# Autodesk Inventor assembly: WheelAssembly
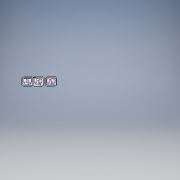
[picture p0: Inventor's stored thumbnail of the model, 180x180]
Saved by Autodesk Inventor 2016 (Build 200138000, 138)
## iProperties
Created: 2016-09-10
Part Number: WheelAssembly
Document SubType Name: Assembly
Designer: RoboticsUser
Author: RoboticsUser
## Documents named in this file (10)
- C:\Robotics\2016-17_CAD\WheelAssembly.iam
- C:\Robotics\CAD\2015-16\custom cad parts\am-2648_4inWheel8mmHub.ipt
- C:\Robotics\CAD\2015-16\COTSParts\Actobotics\545 parts\545556.ipt
- C:\Robotics\CAD\2015-16\COTSParts\Actobotics\615 parts\615102.ipt
- C:\Robotics\CAD\2015-16\COTSParts\Actobotics\634 parts\634080.ipt
- C:\Users\RoboticsUser\Desktop\2015-16 CAD\COTSParts\Actobotics\am-2964NeveRest.ipt
- C:\Users\RoboticsUser\Desktop\2015-16 CAD\COTSParts\Actobotics\615 parts\615114.ipt
- C:\Users\RoboticsUser\Desktop\2015-16 CAD\COTSParts\Tetrix\tetrix-motor-mounts-1.snapshot.1\Tetrex 2pc motor mount.ipt
- C:\Robotics\2016-17_CAD\DriveTrainPlate.iam
- C:\Robotics\CAD\2015-16\COTSParts\Actobotics\545 parts\545456.ipt
## Components (25 placed, 9 different names)
1. am-2648_4inWheel8mmHub:2 — Insert:45, Insert:49
2. 545556:2 — Insert:9, Insert:48, Insert:51
3. 634080:1
4. 615102:3
5. 615102:4 — Insert:44, Mate:1, Angle:1
6. 634080:2 — Insert:9, Insert:41, Insert:47
7. am-2648_4inWheel8mmHub:3 — Insert:12, Insert:14
8. 545556:6 — Insert:12, Insert:50, Insert:52
9. 615102:5
10. 545556:7 — Insert:14
11. 634080:3 — Insert:40, Insert:46
12. am-2964NeveRest:2 — Insert:23, Insert:27
13. 545556:8 — Insert:19, Insert:23
14. 615114:2 — Insert:19
15. 615114:3 — Insert:18
16. 545556:9 — Insert:18, Insert:26
17. am-2964NeveRest:3 — Insert:26, Insert:28
18. Tetrex 2pc motor mount:1 — Insert:27, Insert:31, Insert:32, Insert:33
19. Tetrex 2pc motor mount:2 — Insert:28, Insert:34, Insert:35
20. DriveTrainPlate:1 [sub-assembly] — Insert:31, Insert:32, Insert:33, Insert:34, Insert:35, Insert:46, Insert:47
21. DriveTrainPlate:2 [sub-assembly] — Insert:40, Insert:41, Insert:51, Insert:52
22. 545556:10 — Insert:44, Insert:45
23. 545456:1 — Insert:49, Insert:48
24. 545456:2
25. 545456:3 — Insert:50
## Relationships (29: Insert 27, Mate 1, Angle 1)
- Insert:9 (-12.7 mm): 545556:2 ↔ 634080:2
- Insert:12 (6.35 mm): am-2648_4inWheel8mmHub:3 ↔ 545556:6
- [Insert] (-12.7 mm): 545556:6 ↔ 634080:3
- Insert:14 (9.525 mm): am-2648_4inWheel8mmHub:3 ↔ 545556:7
- [Insert] (2.54 mm): 615102:5 ↔ 545556:7
- Insert:18: 615114:3 ↔ 545556:9
- Insert:19: 545556:8 ↔ 615114:2
- Insert:23 (16.51 mm): am-2964NeveRest:2 ↔ 545556:8
- Insert:26 (16.51 mm): 545556:9 ↔ am-2964NeveRest:3
- Insert:27: am-2964NeveRest:2 ↔ Tetrex 2pc motor mount:1
- Insert:28: am-2964NeveRest:3 ↔ Tetrex 2pc motor mount:2
- Insert:31: Tetrex 2pc motor mount:1 ↔ DriveTrainPlate:1
- Insert:32: Tetrex 2pc motor mount:1 ↔ DriveTrainPlate:1
- Insert:33: Tetrex 2pc motor mount:1 ↔ DriveTrainPlate:1
- Insert:34: Tetrex 2pc motor mount:2 ↔ DriveTrainPlate:1
- Insert:35: Tetrex 2pc motor mount:2 ↔ DriveTrainPlate:1
- Insert:40: 634080:3 ↔ DriveTrainPlate:2
- Insert:41: 634080:2 ↔ DriveTrainPlate:2
- Insert:44: 615102:4 ↔ 545556:10
- Insert:45 (9.525 mm): am-2648_4inWheel8mmHub:2 ↔ 545556:10
- Mate:1: 615102:4
- Angle:1 (0 deg): 615102:4
- Insert:46 (2.3368 mm): 634080:3 ↔ DriveTrainPlate:1
- Insert:47 (2.3368 mm): 634080:2 ↔ DriveTrainPlate:1
- Insert:48: 545556:2 ↔ 545456:1
- Insert:49: am-2648_4inWheel8mmHub:2 ↔ 545456:1
- Insert:50: 545556:6 ↔ 545456:3
- Insert:51 (9.525 mm): 545556:2 ↔ DriveTrainPlate:2
- Insert:52 (9.525 mm): 545556:6 ↔ DriveTrainPlate:2
## Named parameters: d32_d31 = 2.54 mm, d33_d17 = 6.35 mm, d34_d28 = -12.7 mm, d35_d29 = 9.525 mm
